# Autodesk Inventor assembly: NewChassis
(part 2 of 2)
- Mate:652: feeder_guide_plate:1 ↔ PURCHASED,HEX_BEARING:3
- Mate:653: feeder_guide_plate:1 ↔ PURCHASED,HEX_BEARING:3
- Flush:353: am-5123 5IN 500IN Hex Bore Compliant Star:2 ↔ am-5123 5IN 500IN Hex Bore Compliant Star:3
- Mate:654: am-5123 5IN 500IN Hex Bore Compliant Star:2 ↔ 2_1-2_hex_shaft:5
- Mate:655: am-5123 5IN 500IN Hex Bore Compliant Star:2 ↔ 2_1-2_hex_shaft:5
- Mate:656: feeder_bottom_plate:1 ↔ PURCHASED,HEX_BEARING:10
- Mate:657: feeder_bottom_plate:1 ↔ PURCHASED,HEX_BEARING:10
- Mate:658: feeder_bottom_plate:1 ↔ PURCHASED,HEX_BEARING:9
- Mate:659: feeder_bottom_plate:1 ↔ PURCHASED,HEX_BEARING:9
- Mate:660: feeder_guide_plate_MIR:1 ↔ PURCHASED,HEX_BEARING:5
- Mate:661: feeder_guide_plate_MIR:1 ↔ PURCHASED,HEX_BEARING:5
- Mate:662: feeder_guide_plate_MIR:1 ↔ PURCHASED,HEX_BEARING:6
- Mate:663: feeder_guide_plate_MIR:1 ↔ PURCHASED,HEX_BEARING:6
- Mate:664: feeder_guide_plate_MIR:1 ↔ PURCHASED,HEX_BEARING:11
- Mate:665: feeder_guide_plate_MIR:1 ↔ PURCHASED,HEX_BEARING:11
- Mate:666: am-5123 5IN 500IN Hex Bore Compliant Star:7 ↔ 2_1-2_hex_shaft:6
- Mate:667: am-5123 5IN 500IN Hex Bore Compliant Star:7 ↔ 2_1-2_hex_shaft:6
- Flush:354: am-5123 5IN 500IN Hex Bore Compliant Star:2 ↔ am-5123 5IN 500IN Hex Bore Compliant Star:7
- Rotation:1 [RelateRotation] (1 ul): 2_1-2_hex_shaft:3 ↔ 2_1-2_hex_shaft:6
- Rotation:2 [RelateRotation] (1 ul): 2_1-2_hex_shaft:3 ↔ 2_1-2_hex_shaft:4
- Rotation:3 [RelateRotation] (1 ul): 2_1-2_hex_shaft:5 ↔ 2_1-2_hex_shaft:6
- Rotation:4 [RelateRotation] (1 ul): 2_1-2_hex_shaft:1 ↔ 2_1-2_hex_shaft:5
- Rotation:5 [RelateRotation] (1 ul): 2_1-2_hex_shaft:1 ↔ 2_1-2_hex_shaft:2
- Mate:668: VersaPlanetary v2 Dual Stage 10_1 with RS 550 (1):3 ↔ 16t 9mm:2
- Mate:670: VersaPlanetary v2 Dual Stage 10_1 with RS 550 (1):3 ↔ 16t 9mm:2
- Mate:671: 2_1-2_hex_shaft:5 ↔ 16t 9mm:1
- Mate:672: 2_1-2_hex_shaft:5 ↔ 16t 9mm:1
- Flush:355: 16t 9mm:1 ↔ 16t 9mm:2
- Mate:673: VersaPlanetary v2 Dual Stage 10_1 with RS 550 (1):4 ↔ 16t 9mm:3
- Mate:674: VersaPlanetary v2 Dual Stage 10_1 with RS 550 (1):4 ↔ 16t 9mm:3
- Flush:356: 16t 9mm:2 ↔ 16t 9mm:3
- Mate:675: 2_1-2_hex_shaft:6 ↔ 16t 9mm:4
- Mate:676: 2_1-2_hex_shaft:6 ↔ 16t 9mm:4
- Flush:357: 16t 9mm:3 ↔ 16t 9mm:4
- Mate:678: 2_1-2_hex_shaft:6 ↔ 19t 9mm:3
- Mate:677: 16t 9mm:4 ↔ 19t 9mm:3
- Mate:679: 2_1-2_hex_shaft:6 ↔ 19t 9mm:3
- Mate:680: 2_1-2_hex_shaft:3 ↔ 19t 9mm:2
- Flush:358: 19t 9mm:2 ↔ 19t 9mm:3
- Mate:681: 2_1-2_hex_shaft:3 ↔ 19t 9mm:2
- Mate:682: 2_1-2_hex_shaft:5 ↔ 19t 9mm:1
- Mate:683: 16t 9mm:1 ↔ 19t 9mm:1
- Mate:684: 2_1-2_hex_shaft:5 ↔ 19t 9mm:1
- Mate:685: 2_1-2_hex_shaft:1 ↔ 19t 9mm:4
- Flush:359: 19t 9mm:1 ↔ 19t 9mm:4
- Mate:686: 2_1-2_hex_shaft:1 ↔ 19t 9mm:4
- Mate:687: 19t 9mm:4 ↔ 29t 9mm:2
- Mate:688: 2_1-2_hex_shaft:1 ↔ 29t 9mm:2
- Mate:689: 2_1-2_hex_shaft:1 ↔ 29t 9mm:2
- Flush:360: 29t 9mm:1 ↔ 29t 9mm:2
- Mate:690: 2_1-2_hex_shaft:2 ↔ 29t 9mm:1
- Mate:691: 2_1-2_hex_shaft:2 ↔ 29t 9mm:1
- Mate:692: 19t 9mm:2 ↔ 29t 9mm:3
- Mate:693: 2_1-2_hex_shaft:3 ↔ 29t 9mm:3
- Mate:694: 2_1-2_hex_shaft:3 ↔ 29t 9mm:3
- Flush:361: 29t 9mm:3 ↔ 29t 9mm:4
- Mate:695: 2_1-2_hex_shaft:4 ↔ 29t 9mm:4
- Mate:696: 2_1-2_hex_shaft:4 ↔ 29t 9mm:4
- Mate:697: PURCHASED,HEX_BEARING:14 ↔ 16t 9mm:4
- Mate:698: feeder_bottom_plate:1 ↔ Bolt_Spacer:3
- Mate:699: feeder_guide_plate:1 ↔ Bolt_Spacer:3
- Mate:700: feeder_bottom_plate:1 ↔ Bolt_Spacer:4
- Mate:701: feeder_guide_plate_MIR:1 ↔ Bolt_Spacer:4
- Mate:704: coral_end_stop:1 ↔ feeder_front_support:1
- Flush:362 (28.575 mm): coral_end_stop:1 ↔ feeder_front_support:1
- Flush:364: coral_end_stop_MIR:1 ↔ coral_end_stop:1
- Mate:713: Part Studio 1 - Support 1:1 ↔ hopper_side_r:1
- Mate:714: PLATE,BRACE,HORISONTAL,TOP,ELEVATOR.ipt:1 ↔ Part Studio 1 - Support 1:1
- Mate:715 (69.85 mm): coral_end_stop_MIR:1 ↔ coral_end_stop:1
- Flush:365: coral_end_stop_MIR:1 ↔ coral_end_stop:1
- Mate:716: coral_end_stop:1 ↔ feeder_front_support:1
- Mate:717: am-3480 4IN 500Hex Bore Compliant Wheel REV2(1):1 ↔ 2_1-2_hex_shaft:2
- Mate:718: am-3480 4IN 500Hex Bore Compliant Wheel REV2(1):1 ↔ 2_1-2_hex_shaft:2
- Mate:719: am-3480 4IN 500Hex Bore Compliant Wheel REV2(1):1 ↔ PURCHASED,HEX_BEARING:4
- Mate:720: am-3480 4IN 500Hex Bore Compliant Wheel REV2(1):2 ↔ 2_1-2_hex_shaft:4
- Mate:721: am-3480 4IN 500Hex Bore Compliant Wheel REV2(1):2 ↔ 2_1-2_hex_shaft:4
- Mate:722: am-3480 4IN 500Hex Bore Compliant Wheel REV2(1):2 ↔ PURCHASED,HEX_BEARING:6
- Mate:723: 1-2in_spacer:1 ↔ 2_1-2_hex_shaft:2
- Mate:724: 1-2in_spacer:1 ↔ 2_1-2_hex_shaft:2
- Mate:725: am-3480 4IN 500Hex Bore Compliant Wheel REV2(1):1 ↔ 1-2in_spacer:1
- Mate:726: 1-2in_spacer:2 ↔ 2_1-2_hex_shaft:1
- Mate:727: 1-2in_spacer:2 ↔ 2_1-2_hex_shaft:1
- Mate:728: 1-2in_spacer:2 ↔ 19t 9mm:4
- Mate:729: 1-2in_spacer:3 ↔ 2_1-2_hex_shaft:5
- Mate:730: 1-2in_spacer:3 ↔ 2_1-2_hex_shaft:5
- Mate:731: 1-2in_spacer:3 ↔ am-5123 5IN 500IN Hex Bore Compliant Star:2
- Mate:732: 1-2in_spacer:6 ↔ 2_1-2_hex_shaft:6
- Mate:733: 1-2in_spacer:6 ↔ 2_1-2_hex_shaft:6
- Mate:734: 1-2in_spacer:6 ↔ 19t 9mm:3
- Mate:735: 1-2in_spacer:5 ↔ 2_1-2_hex_shaft:3
- Mate:736: 1-2in_spacer:5 ↔ 2_1-2_hex_shaft:3
- Mate:737: 1-2in_spacer:5 ↔ 19t 9mm:2
- Mate:738: 1-2in_spacer:4 ↔ 2_1-2_hex_shaft:4
- Mate:739: 1-2in_spacer:4 ↔ 2_1-2_hex_shaft:4
- Mate:740: 1-2in_spacer:4 ↔ 29t 9mm:4
- Mate:741: feeder_bottom_plate:1 ↔ feeder_guide_plate_MIR:1
- Mate:742: feeder_bottom_plate:1 ↔ feeder_guide_plate:1
- Mate:743: Part Studio 1 - Support 2:1 ↔ hopper_side_l:1
- Mate:744: Part Studio 1 - Support 2:1 ↔ hopper_side_l:1
- Mate:745: Part Studio 1 - Support 2:1 ↔ hopper_side_l:1
- Mate:746: PLATE,BRACE,HORISONTAL,TOP,ELEVATOR.ipt:1 ↔ hopper_backboard:1
- Mate:747: PLATE,BRACE,HORISONTAL,TOP,ELEVATOR.ipt:1 ↔ hopper_backboard:1
- Mate:748: PLATE,BRACE,HORISONTAL,TOP,ELEVATOR.ipt:1 ↔ hopper_backboard:1
- Mate:749: hopper_fin:1 ↔ hopper_back:1
- Mate:750: hopper_fin:1 ↔ hopper_back:1
- Mate:751: hopper_fin_MIR:1 ↔ hopper_back:1
- Mate:752: hopper_fin_MIR:1 ↔ hopper_back:1
- Mate:753: hopper_fin_MIR:1 ↔ hopper_back:1
- Mate:754: hopper_fin:1 ↔ hopper_back:1
## Named parameters: d160_d155 = 0 mm, d161_d156 = 0 mm, d162_d157 = 0 mm, d163_d155 = 0 mm, d164_d156 = 0 mm, d165_d157 = 0 mm, d166_d155 = 0 mm, d167_d156 = 0 mm, d168_d157 = 0 mm, d169_d155 = 0 mm, d170_d156 = 0 mm, d171_d157 = 0 mm, d172_d155 = 0 mm, d173_d156 = 0 mm, d174_d157 = 0 mm, d175_d155 = 0 mm, d176_d156 = 0 mm, d177_d157 = 0 mm, d178_d155 = 0 mm, d179_d156 = 0 mm, d180_d157 = 0 mm, d518_d513 = 0 mm, d875_d873 = 0 mm, d876_d874 = 0 mm, d967_d875_d873 = 0 mm, d968_d876_d874 = 0 mm, d1153_d967_d875_d873 = 0 mm, d1154_d968_d876_d874 = 0 mm, d1199_d1196 = 0 mm, d1200_d1197 = 0 mm, d1201_d1198 = 0 mm, d1224_d1196 = 0 mm, d1225_d1197 = 0 mm, d1226_d1198 = 0 mm, d1227_d1203 = 0 mm, d1228_d1204 = 0 mm, d1233_d1218 = 0 mm, d1237_d1199_d1196 = 0 mm, d1238_d1200_d1197 = 0 mm, d1239_d1201_d1198 = 0 mm, d1249_d1153_d967_d875_d873 = 0 mm, d1250_d1154_d968_d876_d874 = 0 mm, d1274_d169_d155 = 0 mm, d1275_d170_d156 = 0 mm, d1276_d171_d157 = 0 mm, d1277_d169_d155 = 0 mm, d1278_d170_d156 = 0 mm, d1279_d171_d157 = 0 mm
